# Autodesk Inventor assembly: Trebuchet
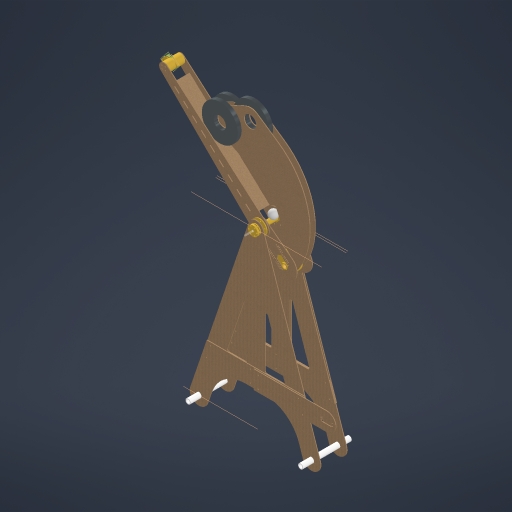
[picture p0: Inventor's stored thumbnail of the model, 512x512]
Saved by Autodesk Inventor 2024.1 (Build 281209000, 209)
## iProperties
Created: 2023-10-16
Part Number: Trebuchet
Document SubType Name: Assembly
Designer: Brandon
Mass: 8239.36 g
Surface Area: 22563.1 cm^2
Volume: 4163.87 cm^3
Density: 1.97877 g/cm^3
Author: Brandon
## Documents named in this file (32)
- C:\Users\Brandon\Documents\School\FallCAD\Trebuchet\Trebuchet\Trebuchet.iam
- C:\Users\Brandon\Documents\School\FallCAD\Trebuchet\Trebuchet\96405K74_Multipurpose Neoprene Rubber Ball\96405K74_Multipurpose Neoprene Rubber Ball.ipt
- C:\Users\Brandon\Documents\School\FallCAD\Trebuchet\Trebuchet\BallBearing_8x22x7mm.ipt
- C:\Users\Brandon\Documents\School\FallCAD\Trebuchet\Trebuchet\AcrylicRod.ipt
- C:\Users\Brandon\Documents\School\FallCAD\Trebuchet\Trebuchet\ArmPivot.ipt
- C:\Users\Brandon\Documents\School\FallCAD\Trebuchet\Trebuchet\ArmPivot2.ipt
- C:\Users\Brandon\Documents\School\FallCAD\Trebuchet\Trebuchet\MainArm.ipt
- C:\Users\Brandon\Documents\School\FallCAD\Trebuchet\Trebuchet\CarabinerThrowMount.ipt
- C:\Users\Brandon\Documents\School\FallCAD\Trebuchet\Trebuchet\94180A351_Tapered Heat-Set Inserts for Plastic\94180A351_Tapered Heat-Set Inserts for Plastic.ipt
- C:\Users\Brandon\Documents\School\FallCAD\Trebuchet\Trebuchet\WeightArm.ipt
- C:\Users\Brandon\Documents\School\FallCAD\Trebuchet\Trebuchet\WeightMount.ipt
- C:\Users\Brandon\Documents\School\FallCAD\Trebuchet\Trebuchet\WeightBearingMount.ipt
- C:\Users\Brandon\Documents\School\FallCAD\Trebuchet\Trebuchet\WeightBearingMount_MIR.ipt
- C:\Users\Brandon\Documents\School\FallCAD\Trebuchet\Trebuchet\LineupSketch.ipt
- C:\Users\Brandon\Documents\School\FallCAD\Trebuchet\Trebuchet\WhipperArm.ipt
- C:\Users\Brandon\Documents\School\FallCAD\Trebuchet\Trebuchet\CounterweightPlate.ipt
- C:\Users\Brandon\Documents\School\FallCAD\Trebuchet\Trebuchet\MainArmCenter.ipt
- C:\Users\Brandon\Documents\School\FallCAD\Trebuchet\Trebuchet\FrameTop.ipt
- C:\Users\Brandon\Documents\School\FallCAD\Trebuchet\Trebuchet\FrameLeg.ipt
- C:\Users\Brandon\Documents\School\FallCAD\Trebuchet\Trebuchet\FrameAxlePVC.ipt
- C:\Users\Brandon\Documents\School\FallCAD\Trebuchet\Trebuchet\MainInnerBearingMount.ipt
- C:\Users\Brandon\Documents\School\FallCAD\Trebuchet\Trebuchet\MainOuterBearingMount.ipt
- C:\Users\Brandon\Documents\School\FallCAD\Trebuchet\Trebuchet\8mmspacer.ipt
- C:\Users\Brandon\Documents\School\FallCAD\Trebuchet\Trebuchet\NewPivotBearingMount.ipt
- C:\Users\Brandon\Documents\School\FallCAD\Trebuchet\Trebuchet\Axle3dprinted.ipt
- C:\Users\Brandon\Documents\School\FallCAD\Trebuchet\Trebuchet\TPUspacer.ipt
- C:\Users\Brandon\Documents\School\FallCAD\Trebuchet\Trebuchet\AxleAdapter.ipt
- C:\Users\Brandon\Documents\School\FallCAD\Trebuchet\Trebuchet\ReleasePin.ipt
- C:\Users\Brandon\Documents\School\FallCAD\Trebuchet\Trebuchet\DropBar.ipt
- C:\Users\Brandon\Documents\School\FallCAD\Trebuchet\Trebuchet\DropBarJoint.ipt
- D:\ServoMount.ipt
- C:\Users\Brandon\Documents\School\FallCAD\Trebuchet\Trebuchet\TrebM4Spacer.ipt
## Components (61 placed, 31 different names)
1. 96405K74_Multipurpose Neoprene Rubber Ball:1
2. BallBearing_8x22x7mm:1 — Insert:1, Flush:1, Flush:2, Insert:19, Flush:14
3. BallBearing_8x22x7mm:2 — Insert:1, Insert:2, Insert:20
4. AcrylicRod:1 — Insert:2
5. ArmPivot:1 — Flush:1, Flush:2, Insert:3, Flush:3
6. ArmPivot2:1 — Insert:3, Insert:4
7. MainArm:1 — Flush:3, Flush:5, Insert:21
8. MainArm:2 — Insert:4, Flush:4, Mate:3, Insert:24, Insert:26, Flush:13, Mate:5, Mate:6
9. CarabinerThrowMount:1 — Flush:4, Flush:22
10. 94180A351_Tapered Heat-Set Inserts for Plastic:1
11. 94180A351_Tapered Heat-Set Inserts for Plastic:2
12. 94180A351_Tapered Heat-Set Inserts for Plastic:3 — Insert:21
13. 94180A351_Tapered Heat-Set Inserts for Plastic:4
14. 94180A351_Tapered Heat-Set Inserts for Plastic:5
15. 94180A351_Tapered Heat-Set Inserts for Plastic:6
16. 94180A351_Tapered Heat-Set Inserts for Plastic:7
17. 94180A351_Tapered Heat-Set Inserts for Plastic:8 — Insert:26
18. WeightArm:1 — Flush:5, Flush:6, Mate:1, Mate:2, Insert:22
19. WeightMount:1 — Flush:6, Mate:1, Mate:2, Insert:13, Insert:15, Insert:22, Insert:25, Insert:28
20. BallBearing_8x22x7mm:3 — Insert:13, Insert:17
21. WeightArm:2 — Mate:3, Insert:24, Insert:25
22. BallBearing_8x22x7mm:4 — Insert:15, Insert:16
23. BallBearing_8x22x7mm:5 — Insert:17, Symmetry:1
24. BallBearing_8x22x7mm:6 — Insert:16, Symmetry:1
25. WeightBearingMount:1 — Flush:7, Flush:8, Insert:18, Angle:2, Angle:3, Insert:27
26. WeightBearingMount_MIR:1 — Flush:9, Flush:10, Flush:12, Insert:23, Angle:2, Insert:27, Insert:28
27. LineupSketch:1 — Flush:11
28. WhipperArm:1 — Flush:12, Insert:23, Angle:1, Insert:29, Insert:31
29. WhipperArm:2 — Insert:18, Angle:1, Angle:3, Insert:30
30. BallBearing_8x22x7mm:7 — Insert:19
31. BallBearing_8x22x7mm:8 — Insert:20
32. CounterweightPlate:1 — Insert:29
33. CounterweightPlate:2 — Insert:30
34. CounterweightPlate:4 — Insert:31
35. MainArmCenter:1 — Flush:13, Mate:5, Mate:6
36. FrameTop:1 — Flush:14, Flush:15, Mate:4, Insert:32, Insert:33, Flush:16
37. FrameLeg:1 — Flush:15
38. FrameLeg:2 — Insert:36, Insert:37, Insert:42
39. FrameLeg:3 — Insert:38, Insert:39
40. FrameLeg:4 — Mate:4, Insert:32, Insert:33, Flush:24, Flush:25
41. FrameTop:2 — Insert:36, Insert:37, Insert:38, Insert:39, Angle:4, Insert:44
42. FrameTop:3 — Flush:17, Mate:12
43. FrameTop:4 — Angle:4, Insert:43
44. FrameAxlePVC:1
45. FrameAxlePVC:2 — Insert:42
46. MainInnerBearingMount:1 — Flush:16
47. MainOuterBearingMount:1 — Flush:17
48. MainOuterBearingMount:2 — Insert:43
49. MainInnerBearingMount:2 — Insert:44
50. 8mmspacer:1
51. FrameTop:5 — Flush:19
52. BallBearing_8x22x7mm:10 — Mate:7, Flush:20
53. NewPivotBearingMount:1 — Flush:19, Flush:21
54. Axle3dprinted:1
55. TPUspacer:1
56. AxleAdapter:1
57. ReleasePin:1 — Flush:22
58. DropBar:1 — Flush:23
59. DropBarJoint:1 — Flush:23
60. ServoMount:1 — Mate:12, Flush:24, Flush:25
61. TrebM4Spacer:1
## Relationships (72: Insert 31, Flush 24, Mate 11, Angle 5, Symmetry 1)
- Insert:1 (100 mm): BallBearing_8x22x7mm:1 ↔ BallBearing_8x22x7mm:2
- Insert:2 (-50 mm): BallBearing_8x22x7mm:2 ↔ AcrylicRod:1
- Flush:1: BallBearing_8x22x7mm:1 ↔ ArmPivot:1
- Flush:2 (10.0076 mm): BallBearing_8x22x7mm:1 ↔ ArmPivot:1
- Insert:3: ArmPivot:1 ↔ ArmPivot2:1
- Flush:3: ArmPivot:1 ↔ MainArm:1
- Insert:4: ArmPivot2:1 ↔ MainArm:2
- Flush:4: MainArm:2 ↔ CarabinerThrowMount:1
- Flush:5: MainArm:1 ↔ WeightArm:1
- Flush:6: WeightArm:1 ↔ WeightMount:1
- Mate:1: WeightArm:1 ↔ WeightMount:1
- Mate:2: WeightArm:1 ↔ WeightMount:1
- Insert:13 (1.27 mm): WeightMount:1 ↔ BallBearing_8x22x7mm:3
- Mate:3: MainArm:2 ↔ WeightArm:2
- Insert:15 (1.27 mm): WeightMount:1 ↔ BallBearing_8x22x7mm:4
- Insert:16: BallBearing_8x22x7mm:4 ↔ BallBearing_8x22x7mm:6
- Insert:17: BallBearing_8x22x7mm:3 ↔ BallBearing_8x22x7mm:5
- Symmetry:1: BallBearing_8x22x7mm:5 ↔ BallBearing_8x22x7mm:6
- Flush:7: WeightBearingMount:1
- Flush:8: WeightBearingMount:1
- Flush:9: WeightBearingMount_MIR:1
- Flush:10: WeightBearingMount_MIR:1
- Flush:11: LineupSketch:1
- Flush:12: WeightBearingMount_MIR:1 ↔ WhipperArm:1
- Insert:18: WeightBearingMount:1 ↔ WhipperArm:2
- Insert:19: BallBearing_8x22x7mm:1 ↔ BallBearing_8x22x7mm:7
- Insert:20: BallBearing_8x22x7mm:2 ↔ BallBearing_8x22x7mm:8
- Insert:21: MainArm:1 ↔ 94180A351_Tapered Heat-Set Inserts for Plastic:3
- Insert:22: WeightArm:1 ↔ WeightMount:1
- Insert:23: WeightBearingMount_MIR:1 ↔ WhipperArm:1
- Angle:1 (0 deg): WhipperArm:1 ↔ WhipperArm:2
- Angle:2 (0 deg): WeightBearingMount:1 ↔ WeightBearingMount_MIR:1
- Angle:3 (0 deg): WeightBearingMount:1 ↔ WhipperArm:2
- Insert:24: MainArm:2 ↔ WeightArm:2
- Insert:25: WeightMount:1 ↔ WeightArm:2
- Insert:26: MainArm:2 ↔ 94180A351_Tapered Heat-Set Inserts for Plastic:8
- Insert:27: WeightBearingMount:1 ↔ WeightBearingMount_MIR:1
- Insert:28 (1.27 mm): WeightMount:1 ↔ WeightBearingMount_MIR:1
- Insert:29: WhipperArm:1 ↔ CounterweightPlate:1
- Insert:30: WhipperArm:2 ↔ CounterweightPlate:2
- Insert:31 (1.524 mm): WhipperArm:1 ↔ CounterweightPlate:4
- Flush:13: MainArm:2 ↔ MainArmCenter:1
- Flush:14: BallBearing_8x22x7mm:1 ↔ FrameTop:1
- Flush:15: FrameTop:1 ↔ FrameLeg:1
- Mate:4: FrameTop:1 ↔ FrameLeg:4
- Insert:32: FrameTop:1 ↔ FrameLeg:4
- Insert:33: FrameTop:1 ↔ FrameLeg:4
- Insert:36: FrameLeg:2 ↔ FrameTop:2
- Insert:37: FrameLeg:2 ↔ FrameTop:2
- Insert:38: FrameLeg:3 ↔ FrameTop:2
- Insert:39: FrameLeg:3 ↔ FrameTop:2
- Angle:4 (0 deg): FrameTop:2 ↔ FrameTop:4
- Mate:5: MainArm:2 ↔ MainArmCenter:1
- Mate:6: MainArm:2 ↔ MainArmCenter:1
- Insert:42 (-45.25 mm): FrameLeg:2 ↔ FrameAxlePVC:2
- Flush:16: FrameTop:1 ↔ MainInnerBearingMount:1
- Flush:17: FrameTop:3 ↔ MainOuterBearingMount:1
- Insert:43: FrameTop:4 ↔ MainOuterBearingMount:2
- Insert:44: FrameTop:2 ↔ MainInnerBearingMount:2
- Mate:7: BallBearing_8x22x7mm:10
- Mate:9
- Mate:10
- Mate:11
- Angle:6 (0 deg)
- Flush:19: FrameTop:5 ↔ NewPivotBearingMount:1
- Flush:20: BallBearing_8x22x7mm:10
- Flush:21: NewPivotBearingMount:1
- Flush:22: CarabinerThrowMount:1 ↔ ReleasePin:1
- Flush:23: DropBar:1 ↔ DropBarJoint:1
- Mate:12: FrameTop:3 ↔ ServoMount:1
- Flush:24: FrameLeg:4 ↔ ServoMount:1
- Flush:25: FrameLeg:4 ↔ ServoMount:1
